# Autodesk Inventor assembly: WedgeBotV2
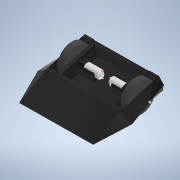
[picture p0: Inventor's stored thumbnail of the model, 180x180]
Saved by Autodesk Inventor 2020 (Build 240168000, 168)
## iProperties
Created: 2023-12-04
Part Number: WedgeBotV2
Document SubType Name: Assembly
Designer: smz3rm
Author: smz3rm
## Documents named in this file (5)
- C:\Users\smz3rm\OneDrive - BP\Documents\DigitalTwin\Models\BattleBot\WedgeBotV2.iam
- C:\Users\smz3rm\OneDrive - BP\Documents\DigitalTwin\Models\BattleBot\BodyWedgeV4.ipt
- C:\Users\smz3rm\OneDrive - BP\Documents\DigitalTwin\Models\BattleBot\DriveMotorV2.ipt
- C:\Users\smz3rm\OneDrive - BP\Documents\DigitalTwin\Models\BattleBot\HubV2.ipt
- C:\Users\smz3rm\OneDrive - BP\Documents\DigitalTwin\Models\BattleBot\WheelV1.ipt
## Components (7 placed, 4 different names)
1. BodyWedgeV4:1 — Mate:4, Mate:5, Mate:6, Mate:7, Mate:8, Mate:9, Mate:10, Mate:14, Mate:15
2. DriveMotorV2:1 — Mate:3, Mate:4, Mate:5, Mate:6
3. HubV2:1 — Mate:1, Mate:2, Mate:3, Mate:7
4. WheelV1:1 — Mate:1, Mate:2
5. DriveMotorV2:2 — Mate:8, Mate:9, Mate:10, Mate:13
6. HubV2:2 — Mate:11, Mate:12, Mate:13, Mate:14
7. WheelV1:2 — Mate:11, Mate:12, Tangent:1
## Relationships (16: Mate 15, Tangent 1)
- Mate:1: HubV2:1 ↔ WheelV1:1
- Mate:2: HubV2:1 ↔ WheelV1:1
- Mate:3: DriveMotorV2:1 ↔ HubV2:1
- Mate:4: BodyWedgeV4:1 ↔ DriveMotorV2:1
- Mate:5: BodyWedgeV4:1 ↔ DriveMotorV2:1
- Mate:6: BodyWedgeV4:1 ↔ DriveMotorV2:1
- Mate:7: BodyWedgeV4:1 ↔ HubV2:1
- Mate:8: BodyWedgeV4:1 ↔ DriveMotorV2:2
- Mate:9: BodyWedgeV4:1 ↔ DriveMotorV2:2
- Mate:10: BodyWedgeV4:1 ↔ DriveMotorV2:2
- Mate:11: HubV2:2 ↔ WheelV1:2
- Mate:12: HubV2:2 ↔ WheelV1:2
- Mate:13: DriveMotorV2:2 ↔ HubV2:2
- Mate:14: BodyWedgeV4:1 ↔ HubV2:2
- Mate:15: BodyWedgeV4:1
- Tangent:1: WheelV1:2
